# Autodesk Inventor assembly: Servo head assembly
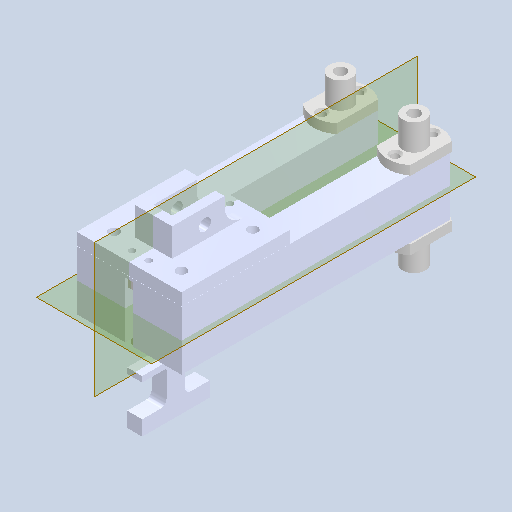
[picture p0: Inventor's stored thumbnail of the model, 512x512]
Saved by Autodesk Inventor 2022 (Build 260153000, 153)
## iProperties
Created: 2021-12-01
Part Number: Servo head assembly
Document SubType Name: Assembly
Designer: efred
Author: efred
## Documents named in this file (8)
- C:\Users\efred\OneDrive - Imperial College London\Old Shit\ROBOICP\Final Assembly\Servo head assembly.iam
- C:\Users\efred\OneDrive - Imperial College London\Old Shit\ROBOICP\Final Assembly\Servo Actuator Mount.ipt
- C:\Users\efred\OneDrive - Imperial College London\Old Shit\ROBOICP\Final Assembly\Linear Bearing.ipt
- C:\Users\efred\OneDrive - Imperial College London\Old Shit\ROBOICP\Final Assembly\Actuator key v2.ipt
- C:\Users\efred\OneDrive - Imperial College London\Old Shit\ROBOICP\Final Assembly\Linear Bearing_MIR2.ipt
- C:\Users\efred\OneDrive - Imperial College London\Old Shit\ROBOICP\Final Assembly\Linear Bearing_MIR3.ipt
- C:\Users\efred\OneDrive - Imperial College London\Old Shit\ROBOICP\Final Assembly\Linear Bearing_MIR2_MIR.ipt
- C:\Users\efred\OneDrive - Imperial College London\Old Shit\ROBOICP\Final Assembly\big servo.ipt
## Components (7 placed, 7 different names)
1. Servo Actuator Mount:1 — Mate:1, Mate:2, Mate:3, Angle:1, Mate:7, Mate:8
2. Linear Bearing:1 — Mate:1, Mate:2, Mate:3
3. Actuator key v2:1 — Mate:4, Mate:5, Angle:1, Mate:9
4. Linear Bearing_MIR2:1
5. Linear Bearing_MIR3:1
6. Linear Bearing_MIR2_MIR:1
7. big servo:1 — Mate:7, Mate:8, Mate:9, Mate:4, Mate:5
## Relationships (9: Mate 8, Angle 1)
- Mate:1: Servo Actuator Mount:1 ↔ Linear Bearing:1
- Mate:2 (0.1 mm): Servo Actuator Mount:1 ↔ Linear Bearing:1
- Mate:3: Servo Actuator Mount:1 ↔ Linear Bearing:1
- Mate:4: Actuator key v2:1 ↔ big servo:1
- Mate:5 (4 mm): Actuator key v2:1 ↔ big servo:1
- Angle:1 (0 deg): Servo Actuator Mount:1 ↔ Actuator key v2:1
- Mate:7 (0.1 mm): Servo Actuator Mount:1 ↔ big servo:1
- Mate:8 (0.1 mm): Servo Actuator Mount:1 ↔ big servo:1
- Mate:9: Actuator key v2:1 ↔ big servo:1
